# Autodesk Inventor assembly: Glock
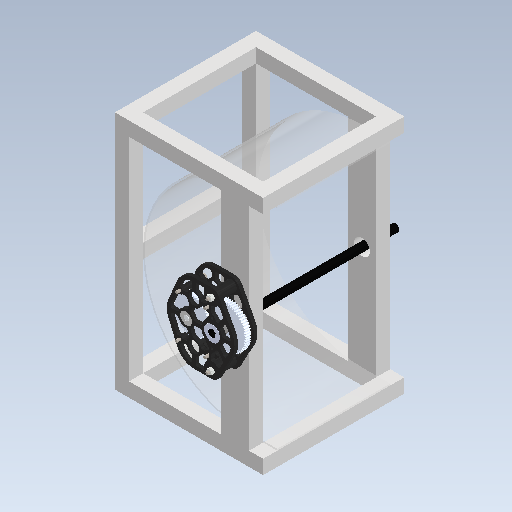
[picture p0: Inventor's stored thumbnail of the model, 512x512]
Saved by Autodesk Inventor 2020 (Build 240168000, 168)
## iProperties
Created: 2020-02-15
Part Number: Glock
Document SubType Name: Assembly
Designer: aidan
Author: aidan
## Documents named in this file (4)
- C:\Users\aidan\Desktop\T3 Robotics\CAD\Glock.iam
- C:\Users\aidan\Desktop\T3 Robotics\CAD\Glock Frame.ipt
- C:\Users\aidan\Desktop\T3 Robotics\CAD\Glock Lexan.ipt
- C:\Users\aidan\Desktop\T3 Robotics\CAD\WCP SS.iam
## Components (3 placed, 3 different names)
1. Glock Frame:1 — Mate:1, Tangent:1, Tangent:2, Flush:1, Mate:2, Mate:3
2. Glock Lexan:1 — Mate:1, Tangent:1, Tangent:2, Flush:1
3. WCP SS:1 [sub-assembly] — Mate:2, Mate:3
## Relationships (6: Mate 3, Tangent 2, Flush 1)
- Mate:1: Glock Frame:1 ↔ Glock Lexan:1
- Tangent:1: Glock Frame:1 ↔ Glock Lexan:1
- Tangent:2: Glock Frame:1 ↔ Glock Lexan:1
- Flush:1: Glock Frame:1 ↔ Glock Lexan:1
- Mate:2: Glock Frame:1 ↔ WCP SS:1
- Mate:3: Glock Frame:1 ↔ WCP SS:1
